# Autodesk Inventor assembly: COMPONENTS
(part 3 of 4)
- C:\Users\rtreacy\Documents\Inventor\SNAP Enclosure 8x10x1.75 Ver1.A\drawings\SNAP Ver2 pack-n-go\Workgroups\NotInProject\INDM9630X305N_L19.ipt
- C:\Users\rtreacy\Documents\Inventor\SNAP Enclosure 8x10x1.75 Ver1.A\drawings\SNAP Ver2 pack-n-go\Workgroups\NotInProject\INDC1608X95L-ALT1_L20.ipt
- C:\Users\rtreacy\Documents\Inventor\SNAP Enclosure 8x10x1.75 Ver1.A\drawings\SNAP Ver2 pack-n-go\Workgroups\NotInProject\INDC1608X95L-ALT1_L21.ipt
- C:\Users\rtreacy\Documents\Inventor\SNAP Enclosure 8x10x1.75 Ver1.A\drawings\SNAP Ver2 pack-n-go\Workgroups\NotInProject\INDC1608X95L-ALT1_L23.ipt
- C:\Users\rtreacy\Documents\Inventor\SNAP Enclosure 8x10x1.75 Ver1.A\drawings\SNAP Ver2 pack-n-go\Workgroups\NotInProject\INDC1608X95L-ALT1_L22.ipt
- C:\Users\rtreacy\Documents\Inventor\SNAP Enclosure 8x10x1.75 Ver1.A\drawings\SNAP Ver2 pack-n-go\Workgroups\NotInProject\INDM5551X200N_L24.ipt
- C:\Users\rtreacy\Documents\Inventor\SNAP Enclosure 8x10x1.75 Ver1.A\drawings\SNAP Ver2 pack-n-go\Workgroups\NotInProject\INDM5551X200N_L25.ipt
- C:\Users\rtreacy\Documents\Inventor\SNAP Enclosure 8x10x1.75 Ver1.A\drawings\SNAP Ver2 pack-n-go\Workgroups\NotInProject\INDM5551X200N_L26.ipt
- C:\Users\rtreacy\Documents\Inventor\SNAP Enclosure 8x10x1.75 Ver1.A\drawings\SNAP Ver2 pack-n-go\Workgroups\NotInProject\INDM5551X200N_L27.ipt
- C:\Users\rtreacy\Documents\Inventor\SNAP Enclosure 8x10x1.75 Ver1.A\drawings\SNAP Ver2 pack-n-go\Workgroups\NotInProject\RESC1005X35N_R443.ipt
- C:\Users\rtreacy\Documents\Inventor\SNAP Enclosure 8x10x1.75 Ver1.A\drawings\SNAP Ver2 pack-n-go\Workgroups\NotInProject\RESC1005X35N_R442.ipt
- C:\Users\rtreacy\Documents\Inventor\SNAP Enclosure 8x10x1.75 Ver1.A\drawings\SNAP Ver2 pack-n-go\Workgroups\NotInProject\RESC1005X35N_R438.ipt
- C:\Users\rtreacy\Documents\Inventor\SNAP Enclosure 8x10x1.75 Ver1.A\drawings\SNAP Ver2 pack-n-go\Workgroups\NotInProject\RESC1005X35N_R437.ipt
- C:\Users\rtreacy\Documents\Inventor\SNAP Enclosure 8x10x1.75 Ver1.A\drawings\SNAP Ver2 pack-n-go\Workgroups\NotInProject\RESC1005X35N_R436.ipt
- C:\Users\rtreacy\Documents\Inventor\SNAP Enclosure 8x10x1.75 Ver1.A\drawings\SNAP Ver2 pack-n-go\Workgroups\NotInProject\RESC1005X35N_R434.ipt
- C:\Users\rtreacy\Documents\Inventor\SNAP Enclosure 8x10x1.75 Ver1.A\drawings\SNAP Ver2 pack-n-go\Workgroups\NotInProject\RESC1005X35N_R114.ipt
- C:\Users\rtreacy\Documents\Inventor\SNAP Enclosure 8x10x1.75 Ver1.A\drawings\SNAP Ver2 pack-n-go\Workgroups\NotInProject\RESC1005X35N_R133.ipt
- C:\Users\rtreacy\Documents\Inventor\SNAP Enclosure 8x10x1.75 Ver1.A\drawings\SNAP Ver2 pack-n-go\Workgroups\NotInProject\RESC1005X35N_R135.ipt
- C:\Users\rtreacy\Documents\Inventor\SNAP Enclosure 8x10x1.75 Ver1.A\drawings\SNAP Ver2 pack-n-go\Workgroups\NotInProject\RESC1005X35N_R139.ipt
- C:\Users\rtreacy\Documents\Inventor\SNAP Enclosure 8x10x1.75 Ver1.A\drawings\SNAP Ver2 pack-n-go\Workgroups\NotInProject\RESC1005X35N_R432.ipt
- C:\Users\rtreacy\Documents\Inventor\SNAP Enclosure 8x10x1.75 Ver1.A\drawings\SNAP Ver2 pack-n-go\Workgroups\NotInProject\RESC1005X35N_R431.ipt
- C:\Users\rtreacy\Documents\Inventor\SNAP Enclosure 8x10x1.75 Ver1.A\drawings\SNAP Ver2 pack-n-go\Workgroups\NotInProject\RESC1005X35N_R427.ipt
- C:\Users\rtreacy\Documents\Inventor\SNAP Enclosure 8x10x1.75 Ver1.A\drawings\SNAP Ver2 pack-n-go\Workgroups\NotInProject\RESC1005X35N_R426.ipt
- C:\Users\rtreacy\Documents\Inventor\SNAP Enclosure 8x10x1.75 Ver1.A\drawings\SNAP Ver2 pack-n-go\Workgroups\NotInProject\RESC1005X35N_R424.ipt
- C:\Users\rtreacy\Documents\Inventor\SNAP Enclosure 8x10x1.75 Ver1.A\drawings\SNAP Ver2 pack-n-go\Workgroups\NotInProject\RESC1005X35N_R423.ipt
- C:\Users\rtreacy\Documents\Inventor\SNAP Enclosure 8x10x1.75 Ver1.A\drawings\SNAP Ver2 pack-n-go\Workgroups\NotInProject\RESC1005X35N_R421.ipt
- C:\Users\rtreacy\Documents\Inventor\SNAP Enclosure 8x10x1.75 Ver1.A\drawings\SNAP Ver2 pack-n-go\Workgroups\NotInProject\RESC1005X35N_R420.ipt
- C:\Users\rtreacy\Documents\Inventor\SNAP Enclosure 8x10x1.75 Ver1.A\drawings\SNAP Ver2 pack-n-go\Workgroups\NotInProject\RESC1005X35N_R433.ipt
- C:\Users\rtreacy\Documents\Inventor\SNAP Enclosure 8x10x1.75 Ver1.A\drawings\SNAP Ver2 pack-n-go\Workgroups\NotInProject\RESC1005X35N_R428.ipt
- C:\Users\rtreacy\Documents\Inventor\SNAP Enclosure 8x10x1.75 Ver1.A\drawings\SNAP Ver2 pack-n-go\Workgroups\NotInProject\RESC1005X35N_R425.ipt
- C:\Users\rtreacy\Documents\Inventor\SNAP Enclosure 8x10x1.75 Ver1.A\drawings\SNAP Ver2 pack-n-go\Workgroups\NotInProject\RESC1005X35N_R422.ipt
- C:\Users\rtreacy\Documents\Inventor\SNAP Enclosure 8x10x1.75 Ver1.A\drawings\SNAP Ver2 pack-n-go\Workgroups\NotInProject\RESC1005X35N_R1.ipt
- C:\Users\rtreacy\Documents\Inventor\SNAP Enclosure 8x10x1.75 Ver1.A\drawings\SNAP Ver2 pack-n-go\Workgroups\NotInProject\RESC1005X35N_R12.ipt
- C:\Users\rtreacy\Documents\Inventor\SNAP Enclosure 8x10x1.75 Ver1.A\drawings\SNAP Ver2 pack-n-go\Workgroups\NotInProject\RESC1005X35N_R13.ipt
- C:\Users\rtreacy\Documents\Inventor\SNAP Enclosure 8x10x1.75 Ver1.A\drawings\SNAP Ver2 pack-n-go\Workgroups\NotInProject\RESC1005X35N_R16.ipt
- C:\Users\rtreacy\Documents\Inventor\SNAP Enclosure 8x10x1.75 Ver1.A\drawings\SNAP Ver2 pack-n-go\Workgroups\NotInProject\RESC1005X35N_R21.ipt
- C:\Users\rtreacy\Documents\Inventor\SNAP Enclosure 8x10x1.75 Ver1.A\drawings\SNAP Ver2 pack-n-go\Workgroups\NotInProject\RESC1005X35N_R25.ipt
- C:\Users\rtreacy\Documents\Inventor\SNAP Enclosure 8x10x1.75 Ver1.A\drawings\SNAP Ver2 pack-n-go\Workgroups\NotInProject\RESC1005X35N_R26.ipt
- C:\Users\rtreacy\Documents\Inventor\SNAP Enclosure 8x10x1.75 Ver1.A\drawings\SNAP Ver2 pack-n-go\Workgroups\NotInProject\RESC1005X35N_R28.ipt
- C:\Users\rtreacy\Documents\Inventor\SNAP Enclosure 8x10x1.75 Ver1.A\drawings\SNAP Ver2 pack-n-go\Workgroups\NotInProject\RESC1005X35N_R29.ipt
- C:\Users\rtreacy\Documents\Inventor\SNAP Enclosure 8x10x1.75 Ver1.A\drawings\SNAP Ver2 pack-n-go\Workgroups\NotInProject\RESC1005X35N_R32.ipt
- C:\Users\rtreacy\Documents\Inventor\SNAP Enclosure 8x10x1.75 Ver1.A\drawings\SNAP Ver2 pack-n-go\Workgroups\NotInProject\RESC1005X35N_R33.ipt
- C:\Users\rtreacy\Documents\Inventor\SNAP Enclosure 8x10x1.75 Ver1.A\drawings\SNAP Ver2 pack-n-go\Workgroups\NotInProject\RESC1005X35N_R36.ipt
- C:\Users\rtreacy\Documents\Inventor\SNAP Enclosure 8x10x1.75 Ver1.A\drawings\SNAP Ver2 pack-n-go\Workgroups\NotInProject\RESC1005X35N_R41.ipt
- C:\Users\rtreacy\Documents\Inventor\SNAP Enclosure 8x10x1.75 Ver1.A\drawings\SNAP Ver2 pack-n-go\Workgroups\NotInProject\RESC1005X35N_R45.ipt
- C:\Users\rtreacy\Documents\Inventor\SNAP Enclosure 8x10x1.75 Ver1.A\drawings\SNAP Ver2 pack-n-go\Workgroups\NotInProject\RESC1005X35N_R46.ipt
- C:\Users\rtreacy\Documents\Inventor\SNAP Enclosure 8x10x1.75 Ver1.A\drawings\SNAP Ver2 pack-n-go\Workgroups\NotInProject\RESC1005X35N_R48.ipt
- C:\Users\rtreacy\Documents\Inventor\SNAP Enclosure 8x10x1.75 Ver1.A\drawings\SNAP Ver2 pack-n-go\Workgroups\NotInProject\RESC1005X35N_R49.ipt
- C:\Users\rtreacy\Documents\Inventor\SNAP Enclosure 8x10x1.75 Ver1.A\drawings\SNAP Ver2 pack-n-go\Workgroups\NotInProject\RESC1005X35N_R5.ipt
- C:\Users\rtreacy\Documents\Inventor\SNAP Enclosure 8x10x1.75 Ver1.A\drawings\SNAP Ver2 pack-n-go\Workgroups\NotInProject\RESC1005X35N_R52.ipt
- C:\Users\rtreacy\Documents\Inventor\SNAP Enclosure 8x10x1.75 Ver1.A\drawings\SNAP Ver2 pack-n-go\Workgroups\NotInProject\RESC1005X35N_R53.ipt
- C:\Users\rtreacy\Documents\Inventor\SNAP Enclosure 8x10x1.75 Ver1.A\drawings\SNAP Ver2 pack-n-go\Workgroups\NotInProject\RESC1005X35N_R56.ipt
- C:\Users\rtreacy\Documents\Inventor\SNAP Enclosure 8x10x1.75 Ver1.A\drawings\SNAP Ver2 pack-n-go\Workgroups\NotInProject\RESC1005X35N_R6.ipt
- C:\Users\rtreacy\Documents\Inventor\SNAP Enclosure 8x10x1.75 Ver1.A\drawings\SNAP Ver2 pack-n-go\Workgroups\NotInProject\RESC1005X35N_R8.ipt
- C:\Users\rtreacy\Documents\Inventor\SNAP Enclosure 8x10x1.75 Ver1.A\drawings\SNAP Ver2 pack-n-go\Workgroups\NotInProject\RESC1005X35N_R9.ipt
- C:\Users\rtreacy\Documents\Inventor\SNAP Enclosure 8x10x1.75 Ver1.A\drawings\SNAP Ver2 pack-n-go\Workgroups\NotInProject\RESC1005X35N_R10.ipt
- C:\Users\rtreacy\Documents\Inventor\SNAP Enclosure 8x10x1.75 Ver1.A\drawings\SNAP Ver2 pack-n-go\Workgroups\NotInProject\RESC1005X35N_R14.ipt
- C:\Users\rtreacy\Documents\Inventor\SNAP Enclosure 8x10x1.75 Ver1.A\drawings\SNAP Ver2 pack-n-go\Workgroups\NotInProject\RESC1005X35N_R2.ipt
- C:\Users\rtreacy\Documents\Inventor\SNAP Enclosure 8x10x1.75 Ver1.A\drawings\SNAP Ver2 pack-n-go\Workgroups\NotInProject\RESC1005X35N_R22.ipt
- C:\Users\rtreacy\Documents\Inventor\SNAP Enclosure 8x10x1.75 Ver1.A\drawings\SNAP Ver2 pack-n-go\Workgroups\NotInProject\RESC1005X35N_R24.ipt
- C:\Users\rtreacy\Documents\Inventor\SNAP Enclosure 8x10x1.75 Ver1.A\drawings\SNAP Ver2 pack-n-go\Workgroups\NotInProject\RESC1005X35N_R30.ipt
- C:\Users\rtreacy\Documents\Inventor\SNAP Enclosure 8x10x1.75 Ver1.A\drawings\SNAP Ver2 pack-n-go\Workgroups\NotInProject\RESC1005X35N_R34.ipt
- C:\Users\rtreacy\Documents\Inventor\SNAP Enclosure 8x10x1.75 Ver1.A\drawings\SNAP Ver2 pack-n-go\Workgroups\NotInProject\RESC1005X35N_R4.ipt
- C:\Users\rtreacy\Documents\Inventor\SNAP Enclosure 8x10x1.75 Ver1.A\drawings\SNAP Ver2 pack-n-go\Workgroups\NotInProject\RESC1005X35N_R42.ipt
- C:\Users\rtreacy\Documents\Inventor\SNAP Enclosure 8x10x1.75 Ver1.A\drawings\SNAP Ver2 pack-n-go\Workgroups\NotInProject\RESC1005X35N_R44.ipt
- C:\Users\rtreacy\Documents\Inventor\SNAP Enclosure 8x10x1.75 Ver1.A\drawings\SNAP Ver2 pack-n-go\Workgroups\NotInProject\RESC1005X35N_R50.ipt
- C:\Users\rtreacy\Documents\Inventor\SNAP Enclosure 8x10x1.75 Ver1.A\drawings\SNAP Ver2 pack-n-go\Workgroups\NotInProject\RESC1005X35N_R54.ipt
- C:\Users\rtreacy\Documents\Inventor\SNAP Enclosure 8x10x1.75 Ver1.A\drawings\SNAP Ver2 pack-n-go\Workgroups\NotInProject\RESC1005X35N_R100.ipt
- C:\Users\rtreacy\Documents\Inventor\SNAP Enclosure 8x10x1.75 Ver1.A\drawings\SNAP Ver2 pack-n-go\Workgroups\NotInProject\RESC1005X35N_R102.ipt
- C:\Users\rtreacy\Documents\Inventor\SNAP Enclosure 8x10x1.75 Ver1.A\drawings\SNAP Ver2 pack-n-go\Workgroups\NotInProject\RESC1005X35N_R103.ipt
- C:\Users\rtreacy\Documents\Inventor\SNAP Enclosure 8x10x1.75 Ver1.A\drawings\SNAP Ver2 pack-n-go\Workgroups\NotInProject\RESC1005X35N_R104.ipt
- C:\Users\rtreacy\Documents\Inventor\SNAP Enclosure 8x10x1.75 Ver1.A\drawings\SNAP Ver2 pack-n-go\Workgroups\NotInProject\RESC1005X35N_R105.ipt
- C:\Users\rtreacy\Documents\Inventor\SNAP Enclosure 8x10x1.75 Ver1.A\drawings\SNAP Ver2 pack-n-go\Workgroups\NotInProject\RESC1005X35N_R106.ipt
- C:\Users\rtreacy\Documents\Inventor\SNAP Enclosure 8x10x1.75 Ver1.A\drawings\SNAP Ver2 pack-n-go\Workgroups\NotInProject\RESC1005X35N_R96.ipt
- C:\Users\rtreacy\Documents\Inventor\SNAP Enclosure 8x10x1.75 Ver1.A\drawings\SNAP Ver2 pack-n-go\Workgroups\NotInProject\RESC1005X35N_R97.ipt
- C:\Users\rtreacy\Documents\Inventor\SNAP Enclosure 8x10x1.75 Ver1.A\drawings\SNAP Ver2 pack-n-go\Workgroups\NotInProject\RESC1005X35N_R109.ipt
- C:\Users\rtreacy\Documents\Inventor\SNAP Enclosure 8x10x1.75 Ver1.A\drawings\SNAP Ver2 pack-n-go\Workgroups\NotInProject\RESC1005X35N_R140.ipt
- C:\Users\rtreacy\Documents\Inventor\SNAP Enclosure 8x10x1.75 Ver1.A\drawings\SNAP Ver2 pack-n-go\Workgroups\NotInProject\RESC1005X35N_R145.ipt
- C:\Users\rtreacy\Documents\Inventor\SNAP Enclosure 8x10x1.75 Ver1.A\drawings\SNAP Ver2 pack-n-go\Workgroups\NotInProject\RESC1005X35N_R146.ipt
- C:\Users\rtreacy\Documents\Inventor\SNAP Enclosure 8x10x1.75 Ver1.A\drawings\SNAP Ver2 pack-n-go\Workgroups\NotInProject\RESC1005X35N_R147.ipt
- C:\Users\rtreacy\Documents\Inventor\SNAP Enclosure 8x10x1.75 Ver1.A\drawings\SNAP Ver2 pack-n-go\Workgroups\NotInProject\RESC1005X35N_R148.ipt
- C:\Users\rtreacy\Documents\Inventor\SNAP Enclosure 8x10x1.75 Ver1.A\drawings\SNAP Ver2 pack-n-go\Workgroups\NotInProject\RESC1005X35N_R154.ipt
- C:\Users\rtreacy\Documents\Inventor\SNAP Enclosure 8x10x1.75 Ver1.A\drawings\SNAP Ver2 pack-n-go\Workgroups\NotInProject\RESC1005X35N_R157.ipt
- C:\Users\rtreacy\Documents\Inventor\SNAP Enclosure 8x10x1.75 Ver1.A\drawings\SNAP Ver2 pack-n-go\Workgroups\NotInProject\RESC1005X35N_R158.ipt
- C:\Users\rtreacy\Documents\Inventor\SNAP Enclosure 8x10x1.75 Ver1.A\drawings\SNAP Ver2 pack-n-go\Workgroups\NotInProject\RESC1005X35N_R159.ipt
- C:\Users\rtreacy\Documents\Inventor\SNAP Enclosure 8x10x1.75 Ver1.A\drawings\SNAP Ver2 pack-n-go\Workgroups\NotInProject\RESC1005X35N_R160.ipt
- C:\Users\rtreacy\Documents\Inventor\SNAP Enclosure 8x10x1.75 Ver1.A\drawings\SNAP Ver2 pack-n-go\Workgroups\NotInProject\RESC1005X35N_R161.ipt
- C:\Users\rtreacy\Documents\Inventor\SNAP Enclosure 8x10x1.75 Ver1.A\drawings\SNAP Ver2 pack-n-go\Workgroups\NotInProject\RESC1005X35N_R162.ipt
- C:\Users\rtreacy\Documents\Inventor\SNAP Enclosure 8x10x1.75 Ver1.A\drawings\SNAP Ver2 pack-n-go\Workgroups\NotInProject\RESC1005X35N_R163.ipt
- C:\Users\rtreacy\Documents\Inventor\SNAP Enclosure 8x10x1.75 Ver1.A\drawings\SNAP Ver2 pack-n-go\Workgroups\NotInProject\RESC1005X35N_R164.ipt
- C:\Users\rtreacy\Documents\Inventor\SNAP Enclosure 8x10x1.75 Ver1.A\drawings\SNAP Ver2 pack-n-go\Workgroups\NotInProject\RESC1005X35N_R194.ipt
- C:\Users\rtreacy\Documents\Inventor\SNAP Enclosure 8x10x1.75 Ver1.A\drawings\SNAP Ver2 pack-n-go\Workgroups\NotInProject\RESC1005X35N_R195.ipt
- C:\Users\rtreacy\Documents\Inventor\SNAP Enclosure 8x10x1.75 Ver1.A\drawings\SNAP Ver2 pack-n-go\Workgroups\NotInProject\RESC1005X35N_R196.ipt
- C:\Users\rtreacy\Documents\Inventor\SNAP Enclosure 8x10x1.75 Ver1.A\drawings\SNAP Ver2 pack-n-go\Workgroups\NotInProject\RESC1005X35N_R201.ipt
- C:\Users\rtreacy\Documents\Inventor\SNAP Enclosure 8x10x1.75 Ver1.A\drawings\SNAP Ver2 pack-n-go\Workgroups\NotInProject\RESC1005X35N_R202.ipt
- C:\Users\rtreacy\Documents\Inventor\SNAP Enclosure 8x10x1.75 Ver1.A\drawings\SNAP Ver2 pack-n-go\Workgroups\NotInProject\RESC1005X35N_R203.ipt
- C:\Users\rtreacy\Documents\Inventor\SNAP Enclosure 8x10x1.75 Ver1.A\drawings\SNAP Ver2 pack-n-go\Workgroups\NotInProject\RESC1005X35N_R204.ipt
- C:\Users\rtreacy\Documents\Inventor\SNAP Enclosure 8x10x1.75 Ver1.A\drawings\SNAP Ver2 pack-n-go\Workgroups\NotInProject\RESC1005X35N_R205.ipt
- C:\Users\rtreacy\Documents\Inventor\SNAP Enclosure 8x10x1.75 Ver1.A\drawings\SNAP Ver2 pack-n-go\Workgroups\NotInProject\RESC1005X35N_R206.ipt
- C:\Users\rtreacy\Documents\Inventor\SNAP Enclosure 8x10x1.75 Ver1.A\drawings\SNAP Ver2 pack-n-go\Workgroups\NotInProject\RESC1005X35N_R207.ipt
- C:\Users\rtreacy\Documents\Inventor\SNAP Enclosure 8x10x1.75 Ver1.A\drawings\SNAP Ver2 pack-n-go\Workgroups\NotInProject\RESC1005X35N_R208.ipt
- C:\Users\rtreacy\Documents\Inventor\SNAP Enclosure 8x10x1.75 Ver1.A\drawings\SNAP Ver2 pack-n-go\Workgroups\NotInProject\RESC1005X35N_R210.ipt
- C:\Users\rtreacy\Documents\Inventor\SNAP Enclosure 8x10x1.75 Ver1.A\drawings\SNAP Ver2 pack-n-go\Workgroups\NotInProject\RESC1005X35N_R211.ipt
- C:\Users\rtreacy\Documents\Inventor\SNAP Enclosure 8x10x1.75 Ver1.A\drawings\SNAP Ver2 pack-n-go\Workgroups\NotInProject\RESC1005X35N_R212.ipt
- C:\Users\rtreacy\Documents\Inventor\SNAP Enclosure 8x10x1.75 Ver1.A\drawings\SNAP Ver2 pack-n-go\Workgroups\NotInProject\RESC1005X35N_R213.ipt
- C:\Users\rtreacy\Documents\Inventor\SNAP Enclosure 8x10x1.75 Ver1.A\drawings\SNAP Ver2 pack-n-go\Workgroups\NotInProject\RESC1005X35N_R214.ipt
- C:\Users\rtreacy\Documents\Inventor\SNAP Enclosure 8x10x1.75 Ver1.A\drawings\SNAP Ver2 pack-n-go\Workgroups\NotInProject\RESC1005X35N_R215.ipt
- C:\Users\rtreacy\Documents\Inventor\SNAP Enclosure 8x10x1.75 Ver1.A\drawings\SNAP Ver2 pack-n-go\Workgroups\NotInProject\RESC1005X35N_R216.ipt
- C:\Users\rtreacy\Documents\Inventor\SNAP Enclosure 8x10x1.75 Ver1.A\drawings\SNAP Ver2 pack-n-go\Workgroups\NotInProject\RESC1005X35N_R217.ipt
- C:\Users\rtreacy\Documents\Inventor\SNAP Enclosure 8x10x1.75 Ver1.A\drawings\SNAP Ver2 pack-n-go\Workgroups\NotInProject\RESC1005X35N_R218.ipt
- C:\Users\rtreacy\Documents\Inventor\SNAP Enclosure 8x10x1.75 Ver1.A\drawings\SNAP Ver2 pack-n-go\Workgroups\NotInProject\RESC1005X35N_R219.ipt
- C:\Users\rtreacy\Documents\Inventor\SNAP Enclosure 8x10x1.75 Ver1.A\drawings\SNAP Ver2 pack-n-go\Workgroups\NotInProject\RESC1005X35N_R221.ipt
- C:\Users\rtreacy\Documents\Inventor\SNAP Enclosure 8x10x1.75 Ver1.A\drawings\SNAP Ver2 pack-n-go\Workgroups\NotInProject\RESC1005X35N_R222.ipt
- C:\Users\rtreacy\Documents\Inventor\SNAP Enclosure 8x10x1.75 Ver1.A\drawings\SNAP Ver2 pack-n-go\Workgroups\NotInProject\RESC1005X35N_R223.ipt
- C:\Users\rtreacy\Documents\Inventor\SNAP Enclosure 8x10x1.75 Ver1.A\drawings\SNAP Ver2 pack-n-go\Workgroups\NotInProject\RESC1005X35N_R224.ipt
- C:\Users\rtreacy\Documents\Inventor\SNAP Enclosure 8x10x1.75 Ver1.A\drawings\SNAP Ver2 pack-n-go\Workgroups\NotInProject\RESC1005X35N_R226.ipt
- C:\Users\rtreacy\Documents\Inventor\SNAP Enclosure 8x10x1.75 Ver1.A\drawings\SNAP Ver2 pack-n-go\Workgroups\NotInProject\RESC1005X35N_R227.ipt
- C:\Users\rtreacy\Documents\Inventor\SNAP Enclosure 8x10x1.75 Ver1.A\drawings\SNAP Ver2 pack-n-go\Workgroups\NotInProject\RESC1005X35N_R11.ipt
- C:\Users\rtreacy\Documents\Inventor\SNAP Enclosure 8x10x1.75 Ver1.A\drawings\SNAP Ver2 pack-n-go\Workgroups\NotInProject\RESC1005X35N_R15.ipt
- C:\Users\rtreacy\Documents\Inventor\SNAP Enclosure 8x10x1.75 Ver1.A\drawings\SNAP Ver2 pack-n-go\Workgroups\NotInProject\RESC1005X35N_R23.ipt
- C:\Users\rtreacy\Documents\Inventor\SNAP Enclosure 8x10x1.75 Ver1.A\drawings\SNAP Ver2 pack-n-go\Workgroups\NotInProject\RESC1005X35N_R27.ipt
- C:\Users\rtreacy\Documents\Inventor\SNAP Enclosure 8x10x1.75 Ver1.A\drawings\SNAP Ver2 pack-n-go\Workgroups\NotInProject\RESC1005X35N_R3.ipt
- C:\Users\rtreacy\Documents\Inventor\SNAP Enclosure 8x10x1.75 Ver1.A\drawings\SNAP Ver2 pack-n-go\Workgroups\NotInProject\RESC1005X35N_R31.ipt
- C:\Users\rtreacy\Documents\Inventor\SNAP Enclosure 8x10x1.75 Ver1.A\drawings\SNAP Ver2 pack-n-go\Workgroups\NotInProject\RESC1005X35N_R35.ipt
- C:\Users\rtreacy\Documents\Inventor\SNAP Enclosure 8x10x1.75 Ver1.A\drawings\SNAP Ver2 pack-n-go\Workgroups\NotInProject\RESC1005X35N_R43.ipt
- C:\Users\rtreacy\Documents\Inventor\SNAP Enclosure 8x10x1.75 Ver1.A\drawings\SNAP Ver2 pack-n-go\Workgroups\NotInProject\RESC1005X35N_R47.ipt
- C:\Users\rtreacy\Documents\Inventor\SNAP Enclosure 8x10x1.75 Ver1.A\drawings\SNAP Ver2 pack-n-go\Workgroups\NotInProject\RESC1005X35N_R51.ipt
- C:\Users\rtreacy\Documents\Inventor\SNAP Enclosure 8x10x1.75 Ver1.A\drawings\SNAP Ver2 pack-n-go\Workgroups\NotInProject\RESC1005X35N_R55.ipt
- C:\Users\rtreacy\Documents\Inventor\SNAP Enclosure 8x10x1.75 Ver1.A\drawings\SNAP Ver2 pack-n-go\Workgroups\NotInProject\RESC1005X35N_R7.ipt
- C:\Users\rtreacy\Documents\Inventor\SNAP Enclosure 8x10x1.75 Ver1.A\drawings\SNAP Ver2 pack-n-go\Workgroups\NotInProject\RESC1005X35N_R110.ipt
- C:\Users\rtreacy\Documents\Inventor\SNAP Enclosure 8x10x1.75 Ver1.A\drawings\SNAP Ver2 pack-n-go\Workgroups\NotInProject\RESC1005X35N_R112.ipt
- C:\Users\rtreacy\Documents\Inventor\SNAP Enclosure 8x10x1.75 Ver1.A\drawings\SNAP Ver2 pack-n-go\Workgroups\NotInProject\RESC1005X35N_R113.ipt
- C:\Users\rtreacy\Documents\Inventor\SNAP Enclosure 8x10x1.75 Ver1.A\drawings\SNAP Ver2 pack-n-go\Workgroups\NotInProject\RESC1005X35N_R115.ipt
- C:\Users\rtreacy\Documents\Inventor\SNAP Enclosure 8x10x1.75 Ver1.A\drawings\SNAP Ver2 pack-n-go\Workgroups\NotInProject\RESC1005X35N_R116.ipt
- C:\Users\rtreacy\Documents\Inventor\SNAP Enclosure 8x10x1.75 Ver1.A\drawings\SNAP Ver2 pack-n-go\Workgroups\NotInProject\RESC1005X35N_R120.ipt
- C:\Users\rtreacy\Documents\Inventor\SNAP Enclosure 8x10x1.75 Ver1.A\drawings\SNAP Ver2 pack-n-go\Workgroups\NotInProject\RESC1005X35N_R124.ipt
- C:\Users\rtreacy\Documents\Inventor\SNAP Enclosure 8x10x1.75 Ver1.A\drawings\SNAP Ver2 pack-n-go\Workgroups\NotInProject\RESC1005X35N_R111.ipt
- C:\Users\rtreacy\Documents\Inventor\SNAP Enclosure 8x10x1.75 Ver1.A\drawings\SNAP Ver2 pack-n-go\Workgroups\NotInProject\RESC1005X35N_R117.ipt
- C:\Users\rtreacy\Documents\Inventor\SNAP Enclosure 8x10x1.75 Ver1.A\drawings\SNAP Ver2 pack-n-go\Workgroups\NotInProject\RESC1005X35N_R119.ipt
- C:\Users\rtreacy\Documents\Inventor\SNAP Enclosure 8x10x1.75 Ver1.A\drawings\SNAP Ver2 pack-n-go\Workgroups\NotInProject\RESC1005X35N_R123.ipt
- C:\Users\rtreacy\Documents\Inventor\SNAP Enclosure 8x10x1.75 Ver1.A\drawings\SNAP Ver2 pack-n-go\Workgroups\NotInProject\RESC1005X35N_R130.ipt
- C:\Users\rtreacy\Documents\Inventor\SNAP Enclosure 8x10x1.75 Ver1.A\drawings\SNAP Ver2 pack-n-go\Workgroups\NotInProject\RESC1005X35N_R132.ipt
- C:\Users\rtreacy\Documents\Inventor\SNAP Enclosure 8x10x1.75 Ver1.A\drawings\SNAP Ver2 pack-n-go\Workgroups\NotInProject\RESC1005X35N_R134.ipt
- C:\Users\rtreacy\Documents\Inventor\SNAP Enclosure 8x10x1.75 Ver1.A\drawings\SNAP Ver2 pack-n-go\Workgroups\NotInProject\RESC1005X35N_R137.ipt
- C:\Users\rtreacy\Documents\Inventor\SNAP Enclosure 8x10x1.75 Ver1.A\drawings\SNAP Ver2 pack-n-go\Workgroups\NotInProject\RESC1005X35N_R170.ipt
- C:\Users\rtreacy\Documents\Inventor\SNAP Enclosure 8x10x1.75 Ver1.A\drawings\SNAP Ver2 pack-n-go\Workgroups\NotInProject\RESC1005X35N_R171.ipt
- C:\Users\rtreacy\Documents\Inventor\SNAP Enclosure 8x10x1.75 Ver1.A\drawings\SNAP Ver2 pack-n-go\Workgroups\NotInProject\RESC1005X35N_R175.ipt
- C:\Users\rtreacy\Documents\Inventor\SNAP Enclosure 8x10x1.75 Ver1.A\drawings\SNAP Ver2 pack-n-go\Workgroups\NotInProject\RESC1005X35N_R178.ipt
- C:\Users\rtreacy\Documents\Inventor\SNAP Enclosure 8x10x1.75 Ver1.A\drawings\SNAP Ver2 pack-n-go\Workgroups\NotInProject\RESC1005X35N_R183.ipt
- C:\Users\rtreacy\Documents\Inventor\SNAP Enclosure 8x10x1.75 Ver1.A\drawings\SNAP Ver2 pack-n-go\Workgroups\NotInProject\RESC1005X35N_R184.ipt
- C:\Users\rtreacy\Documents\Inventor\SNAP Enclosure 8x10x1.75 Ver1.A\drawings\SNAP Ver2 pack-n-go\Workgroups\NotInProject\RESC1005X35N_R188.ipt
- C:\Users\rtreacy\Documents\Inventor\SNAP Enclosure 8x10x1.75 Ver1.A\drawings\SNAP Ver2 pack-n-go\Workgroups\NotInProject\RESC1005X35N_R191.ipt
- C:\Users\rtreacy\Documents\Inventor\SNAP Enclosure 8x10x1.75 Ver1.A\drawings\SNAP Ver2 pack-n-go\Workgroups\NotInProject\RESC1005X35N_R118.ipt
- C:\Users\rtreacy\Documents\Inventor\SNAP Enclosure 8x10x1.75 Ver1.A\drawings\SNAP Ver2 pack-n-go\Workgroups\NotInProject\RESC1005X35N_R121.ipt
- C:\Users\rtreacy\Documents\Inventor\SNAP Enclosure 8x10x1.75 Ver1.A\drawings\SNAP Ver2 pack-n-go\Workgroups\NotInProject\RESC1005X35N_R126.ipt
- C:\Users\rtreacy\Documents\Inventor\SNAP Enclosure 8x10x1.75 Ver1.A\drawings\SNAP Ver2 pack-n-go\Workgroups\NotInProject\RESC1005X35N_R131.ipt
- C:\Users\rtreacy\Documents\Inventor\SNAP Enclosure 8x10x1.75 Ver1.A\drawings\SNAP Ver2 pack-n-go\Workgroups\NotInProject\RESC1005X35N_R122.ipt
- C:\Users\rtreacy\Documents\Inventor\SNAP Enclosure 8x10x1.75 Ver1.A\drawings\SNAP Ver2 pack-n-go\Workgroups\NotInProject\RESC1005X35N_R125.ipt
- C:\Users\rtreacy\Documents\Inventor\SNAP Enclosure 8x10x1.75 Ver1.A\drawings\SNAP Ver2 pack-n-go\Workgroups\NotInProject\RESC1005X35N_R138.ipt
- C:\Users\rtreacy\Documents\Inventor\SNAP Enclosure 8x10x1.75 Ver1.A\drawings\SNAP Ver2 pack-n-go\Workgroups\NotInProject\RESC1005X35N_R127.ipt
- C:\Users\rtreacy\Documents\Inventor\SNAP Enclosure 8x10x1.75 Ver1.A\drawings\SNAP Ver2 pack-n-go\Workgroups\NotInProject\RESC1005X35N_R128.ipt
- C:\Users\rtreacy\Documents\Inventor\SNAP Enclosure 8x10x1.75 Ver1.A\drawings\SNAP Ver2 pack-n-go\Workgroups\NotInProject\RESC1005X35N_R166.ipt
- C:\Users\rtreacy\Documents\Inventor\SNAP Enclosure 8x10x1.75 Ver1.A\drawings\SNAP Ver2 pack-n-go\Workgroups\NotInProject\RESC1005X35N_R167.ipt
- C:\Users\rtreacy\Documents\Inventor\SNAP Enclosure 8x10x1.75 Ver1.A\drawings\SNAP Ver2 pack-n-go\Workgroups\NotInProject\RESC1005X35N_R169.ipt
- C:\Users\rtreacy\Documents\Inventor\SNAP Enclosure 8x10x1.75 Ver1.A\drawings\SNAP Ver2 pack-n-go\Workgroups\NotInProject\RESC1005X35N_R172.ipt
- C:\Users\rtreacy\Documents\Inventor\SNAP Enclosure 8x10x1.75 Ver1.A\drawings\SNAP Ver2 pack-n-go\Workgroups\NotInProject\RESC1005X35N_R173.ipt
- C:\Users\rtreacy\Documents\Inventor\SNAP Enclosure 8x10x1.75 Ver1.A\drawings\SNAP Ver2 pack-n-go\Workgroups\NotInProject\RESC1005X35N_R174.ipt
- C:\Users\rtreacy\Documents\Inventor\SNAP Enclosure 8x10x1.75 Ver1.A\drawings\SNAP Ver2 pack-n-go\Workgroups\NotInProject\RESC1005X35N_R176.ipt
- C:\Users\rtreacy\Documents\Inventor\SNAP Enclosure 8x10x1.75 Ver1.A\drawings\SNAP Ver2 pack-n-go\Workgroups\NotInProject\RESC1005X35N_R177.ipt
- C:\Users\rtreacy\Documents\Inventor\SNAP Enclosure 8x10x1.75 Ver1.A\drawings\SNAP Ver2 pack-n-go\Workgroups\NotInProject\RESC1005X35N_R179.ipt
- C:\Users\rtreacy\Documents\Inventor\SNAP Enclosure 8x10x1.75 Ver1.A\drawings\SNAP Ver2 pack-n-go\Workgroups\NotInProject\RESC1005X35N_R180.ipt
- C:\Users\rtreacy\Documents\Inventor\SNAP Enclosure 8x10x1.75 Ver1.A\drawings\SNAP Ver2 pack-n-go\Workgroups\NotInProject\RESC1005X35N_R182.ipt
- C:\Users\rtreacy\Documents\Inventor\SNAP Enclosure 8x10x1.75 Ver1.A\drawings\SNAP Ver2 pack-n-go\Workgroups\NotInProject\RESC1005X35N_R185.ipt
- C:\Users\rtreacy\Documents\Inventor\SNAP Enclosure 8x10x1.75 Ver1.A\drawings\SNAP Ver2 pack-n-go\Workgroups\NotInProject\RESC1005X35N_R186.ipt
- C:\Users\rtreacy\Documents\Inventor\SNAP Enclosure 8x10x1.75 Ver1.A\drawings\SNAP Ver2 pack-n-go\Workgroups\NotInProject\RESC1005X35N_R187.ipt
- C:\Users\rtreacy\Documents\Inventor\SNAP Enclosure 8x10x1.75 Ver1.A\drawings\SNAP Ver2 pack-n-go\Workgroups\NotInProject\RESC1005X35N_R189.ipt
- C:\Users\rtreacy\Documents\Inventor\SNAP Enclosure 8x10x1.75 Ver1.A\drawings\SNAP Ver2 pack-n-go\Workgroups\NotInProject\RESC1005X35N_R190.ipt
- C:\Users\rtreacy\Documents\Inventor\SNAP Enclosure 8x10x1.75 Ver1.A\drawings\SNAP Ver2 pack-n-go\Workgroups\NotInProject\RESC1005X35N_R136.ipt
- C:\Users\rtreacy\Documents\Inventor\SNAP Enclosure 8x10x1.75 Ver1.A\drawings\SNAP Ver2 pack-n-go\Workgroups\NotInProject\RESC1005X35N_R141.ipt
- C:\Users\rtreacy\Documents\Inventor\SNAP Enclosure 8x10x1.75 Ver1.A\drawings\SNAP Ver2 pack-n-go\Workgroups\NotInProject\RESC1005X35N_R142.ipt
- C:\Users\rtreacy\Documents\Inventor\SNAP Enclosure 8x10x1.75 Ver1.A\drawings\SNAP Ver2 pack-n-go\Workgroups\NotInProject\RESC1005X35N_R143.ipt
- C:\Users\rtreacy\Documents\Inventor\SNAP Enclosure 8x10x1.75 Ver1.A\drawings\SNAP Ver2 pack-n-go\Workgroups\NotInProject\RESC1005X35N_R144.ipt
- C:\Users\rtreacy\Documents\Inventor\SNAP Enclosure 8x10x1.75 Ver1.A\drawings\SNAP Ver2 pack-n-go\Workgroups\NotInProject\RESC1005X35N_R197.ipt
- C:\Users\rtreacy\Documents\Inventor\SNAP Enclosure 8x10x1.75 Ver1.A\drawings\SNAP Ver2 pack-n-go\Workgroups\NotInProject\RESC1005X35N_R198.ipt
- C:\Users\rtreacy\Documents\Inventor\SNAP Enclosure 8x10x1.75 Ver1.A\drawings\SNAP Ver2 pack-n-go\Workgroups\NotInProject\RESC1005X35N_R199.ipt
- C:\Users\rtreacy\Documents\Inventor\SNAP Enclosure 8x10x1.75 Ver1.A\drawings\SNAP Ver2 pack-n-go\Workgroups\NotInProject\RESC1005X35N_R200.ipt
- C:\Users\rtreacy\Documents\Inventor\SNAP Enclosure 8x10x1.75 Ver1.A\drawings\SNAP Ver2 pack-n-go\Workgroups\NotInProject\RESC1005X35N_R155.ipt
- C:\Users\rtreacy\Documents\Inventor\SNAP Enclosure 8x10x1.75 Ver1.A\drawings\SNAP Ver2 pack-n-go\Workgroups\NotInProject\RESC1005X35N_R156.ipt
- C:\Users\rtreacy\Documents\Inventor\SNAP Enclosure 8x10x1.75 Ver1.A\drawings\SNAP Ver2 pack-n-go\Workgroups\NotInProject\RESC1005X35N_R225.ipt
- C:\Users\rtreacy\Documents\Inventor\SNAP Enclosure 8x10x1.75 Ver1.A\drawings\SNAP Ver2 pack-n-go\Workgroups\NotInProject\RESC1005X35N_R228.ipt
- C:\Users\rtreacy\Documents\Inventor\SNAP Enclosure 8x10x1.75 Ver1.A\drawings\SNAP Ver2 pack-n-go\Workgroups\NotInProject\RESC1005X35N_R229.ipt
- C:\Users\rtreacy\Documents\Inventor\SNAP Enclosure 8x10x1.75 Ver1.A\drawings\SNAP Ver2 pack-n-go\Workgroups\NotInProject\RESC1005X35N_R230.ipt
- C:\Users\rtreacy\Documents\Inventor\SNAP Enclosure 8x10x1.75 Ver1.A\drawings\SNAP Ver2 pack-n-go\Workgroups\NotInProject\RESC1005X35N_R231.ipt
- C:\Users\rtreacy\Documents\Inventor\SNAP Enclosure 8x10x1.75 Ver1.A\drawings\SNAP Ver2 pack-n-go\Workgroups\NotInProject\RESC1005X35N_R232.ipt
- C:\Users\rtreacy\Documents\Inventor\SNAP Enclosure 8x10x1.75 Ver1.A\drawings\SNAP Ver2 pack-n-go\Workgroups\NotInProject\RESC1005X35N_R233.ipt
- C:\Users\rtreacy\Documents\Inventor\SNAP Enclosure 8x10x1.75 Ver1.A\drawings\SNAP Ver2 pack-n-go\Workgroups\NotInProject\RESC1005X35N_R234.ipt
- C:\Users\rtreacy\Documents\Inventor\SNAP Enclosure 8x10x1.75 Ver1.A\drawings\SNAP Ver2 pack-n-go\Workgroups\NotInProject\RESC1005X35N_R168.ipt
- C:\Users\rtreacy\Documents\Inventor\SNAP Enclosure 8x10x1.75 Ver1.A\drawings\SNAP Ver2 pack-n-go\Workgroups\NotInProject\RESC1005X35N_R181.ipt
- C:\Users\rtreacy\Documents\Inventor\SNAP Enclosure 8x10x1.75 Ver1.A\drawings\SNAP Ver2 pack-n-go\Workgroups\NotInProject\RESC1005X35N_R17.ipt
- C:\Users\rtreacy\Documents\Inventor\SNAP Enclosure 8x10x1.75 Ver1.A\drawings\SNAP Ver2 pack-n-go\Workgroups\NotInProject\RESC1005X35N_R18.ipt
- C:\Users\rtreacy\Documents\Inventor\SNAP Enclosure 8x10x1.75 Ver1.A\drawings\SNAP Ver2 pack-n-go\Workgroups\NotInProject\RESC1005X35N_R37.ipt
- C:\Users\rtreacy\Documents\Inventor\SNAP Enclosure 8x10x1.75 Ver1.A\drawings\SNAP Ver2 pack-n-go\Workgroups\NotInProject\RESC1005X35N_R38.ipt
- C:\Users\rtreacy\Documents\Inventor\SNAP Enclosure 8x10x1.75 Ver1.A\drawings\SNAP Ver2 pack-n-go\Workgroups\NotInProject\RESC1005X35N_R57.ipt
- C:\Users\rtreacy\Documents\Inventor\SNAP Enclosure 8x10x1.75 Ver1.A\drawings\SNAP Ver2 pack-n-go\Workgroups\NotInProject\RESC1005X35N_R58.ipt
- C:\Users\rtreacy\Documents\Inventor\SNAP Enclosure 8x10x1.75 Ver1.A\drawings\SNAP Ver2 pack-n-go\Workgroups\NotInProject\RESC1005X35N_R19.ipt
- C:\Users\rtreacy\Documents\Inventor\SNAP Enclosure 8x10x1.75 Ver1.A\drawings\SNAP Ver2 pack-n-go\Workgroups\NotInProject\RESC1005X35N_R39.ipt
- C:\Users\rtreacy\Documents\Inventor\SNAP Enclosure 8x10x1.75 Ver1.A\drawings\SNAP Ver2 pack-n-go\Workgroups\NotInProject\RESC1005X35N_R59.ipt
- C:\Users\rtreacy\Documents\Inventor\SNAP Enclosure 8x10x1.75 Ver1.A\drawings\SNAP Ver2 pack-n-go\Workgroups\NotInProject\RESC1005X35N_R20.ipt
- C:\Users\rtreacy\Documents\Inventor\SNAP Enclosure 8x10x1.75 Ver1.A\drawings\SNAP Ver2 pack-n-go\Workgroups\NotInProject\RESC1005X35N_R40.ipt
- C:\Users\rtreacy\Documents\Inventor\SNAP Enclosure 8x10x1.75 Ver1.A\drawings\SNAP Ver2 pack-n-go\Workgroups\NotInProject\RESC1005X35N_R60.ipt
- C:\Users\rtreacy\Documents\Inventor\SNAP Enclosure 8x10x1.75 Ver1.A\drawings\SNAP Ver2 pack-n-go\Workgroups\NotInProject\RESC1005X35N_R209.ipt
- C:\Users\rtreacy\Documents\Inventor\SNAP Enclosure 8x10x1.75 Ver1.A\drawings\SNAP Ver2 pack-n-go\Workgroups\NotInProject\RESC1005X35N_R220.ipt
- C:\Users\rtreacy\Documents\Inventor\SNAP Enclosure 8x10x1.75 Ver1.A\drawings\SNAP Ver2 pack-n-go\Workgroups\NotInProject\RESC1005X35N_R61.ipt
- C:\Users\rtreacy\Documents\Inventor\SNAP Enclosure 8x10x1.75 Ver1.A\drawings\SNAP Ver2 pack-n-go\Workgroups\NotInProject\RESC1005X35N_R65.ipt
- C:\Users\rtreacy\Documents\Inventor\SNAP Enclosure 8x10x1.75 Ver1.A\drawings\SNAP Ver2 pack-n-go\Workgroups\NotInProject\RESC1005X35N_R67.ipt
- C:\Users\rtreacy\Documents\Inventor\SNAP Enclosure 8x10x1.75 Ver1.A\drawings\SNAP Ver2 pack-n-go\Workgroups\NotInProject\RESC1005X35N_R62.ipt
- C:\Users\rtreacy\Documents\Inventor\SNAP Enclosure 8x10x1.75 Ver1.A\drawings\SNAP Ver2 pack-n-go\Workgroups\NotInProject\RESC1005X35N_R64.ipt
- C:\Users\rtreacy\Documents\Inventor\SNAP Enclosure 8x10x1.75 Ver1.A\drawings\SNAP Ver2 pack-n-go\Workgroups\NotInProject\RESC1005X35N_R63.ipt
- C:\Users\rtreacy\Documents\Inventor\SNAP Enclosure 8x10x1.75 Ver1.A\drawings\SNAP Ver2 pack-n-go\Workgroups\NotInProject\RESC1005X35N_R66.ipt
- C:\Users\rtreacy\Documents\Inventor\SNAP Enclosure 8x10x1.75 Ver1.A\drawings\SNAP Ver2 pack-n-go\Workgroups\NotInProject\RESC1005X35N_R70.ipt
- C:\Users\rtreacy\Documents\Inventor\SNAP Enclosure 8x10x1.75 Ver1.A\drawings\SNAP Ver2 pack-n-go\Workgroups\NotInProject\RESC1005X35N_R71.ipt
- C:\Users\rtreacy\Documents\Inventor\SNAP Enclosure 8x10x1.75 Ver1.A\drawings\SNAP Ver2 pack-n-go\Workgroups\NotInProject\RESC1005X35N_R72.ipt
- C:\Users\rtreacy\Documents\Inventor\SNAP Enclosure 8x10x1.75 Ver1.A\drawings\SNAP Ver2 pack-n-go\Workgroups\NotInProject\RESC1005X35N_R73.ipt
- C:\Users\rtreacy\Documents\Inventor\SNAP Enclosure 8x10x1.75 Ver1.A\drawings\SNAP Ver2 pack-n-go\Workgroups\NotInProject\RESC1005X35N_R75.ipt
- C:\Users\rtreacy\Documents\Inventor\SNAP Enclosure 8x10x1.75 Ver1.A\drawings\SNAP Ver2 pack-n-go\Workgroups\NotInProject\RESC1005X35N_R76.ipt
- C:\Users\rtreacy\Documents\Inventor\SNAP Enclosure 8x10x1.75 Ver1.A\drawings\SNAP Ver2 pack-n-go\Workgroups\NotInProject\RESC1005X35N_R77.ipt
- C:\Users\rtreacy\Documents\Inventor\SNAP Enclosure 8x10x1.75 Ver1.A\drawings\SNAP Ver2 pack-n-go\Workgroups\NotInProject\RESC1005X35N_R91.ipt
- C:\Users\rtreacy\Documents\Inventor\SNAP Enclosure 8x10x1.75 Ver1.A\drawings\SNAP Ver2 pack-n-go\Workgroups\NotInProject\RESC1005X35N_R92.ipt
- C:\Users\rtreacy\Documents\Inventor\SNAP Enclosure 8x10x1.75 Ver1.A\drawings\SNAP Ver2 pack-n-go\Workgroups\NotInProject\RESC1005X35N_R94.ipt
- C:\Users\rtreacy\Documents\Inventor\SNAP Enclosure 8x10x1.75 Ver1.A\drawings\SNAP Ver2 pack-n-go\Workgroups\NotInProject\RESC1005X35N_R95.ipt
- C:\Users\rtreacy\Documents\Inventor\SNAP Enclosure 8x10x1.75 Ver1.A\drawings\SNAP Ver2 pack-n-go\Workgroups\NotInProject\RESC1005X35N_R80.ipt
- C:\Users\rtreacy\Documents\Inventor\SNAP Enclosure 8x10x1.75 Ver1.A\drawings\SNAP Ver2 pack-n-go\Workgroups\NotInProject\RESC1005X35N_R81.ipt
- C:\Users\rtreacy\Documents\Inventor\SNAP Enclosure 8x10x1.75 Ver1.A\drawings\SNAP Ver2 pack-n-go\Workgroups\NotInProject\RESC1005X35N_R82.ipt
- C:\Users\rtreacy\Documents\Inventor\SNAP Enclosure 8x10x1.75 Ver1.A\drawings\SNAP Ver2 pack-n-go\Workgroups\NotInProject\RESC1005X35N_R83.ipt
- C:\Users\rtreacy\Documents\Inventor\SNAP Enclosure 8x10x1.75 Ver1.A\drawings\SNAP Ver2 pack-n-go\Workgroups\NotInProject\RESC1005X35N_R84.ipt
- C:\Users\rtreacy\Documents\Inventor\SNAP Enclosure 8x10x1.75 Ver1.A\drawings\SNAP Ver2 pack-n-go\Workgroups\NotInProject\RESC1005X35N_R86.ipt
- C:\Users\rtreacy\Documents\Inventor\SNAP Enclosure 8x10x1.75 Ver1.A\drawings\SNAP Ver2 pack-n-go\Workgroups\NotInProject\RESC1005X35N_R90.ipt
- C:\Users\rtreacy\Documents\Inventor\SNAP Enclosure 8x10x1.75 Ver1.A\drawings\SNAP Ver2 pack-n-go\Workgroups\NotInProject\RESC1005X35N_R93.ipt
- C:\Users\rtreacy\Documents\Inventor\SNAP Enclosure 8x10x1.75 Ver1.A\drawings\SNAP Ver2 pack-n-go\Workgroups\NotInProject\RESC1005X35N_R99.ipt
- C:\Users\rtreacy\Documents\Inventor\SNAP Enclosure 8x10x1.75 Ver1.A\drawings\SNAP Ver2 pack-n-go\Workgroups\NotInProject\RESC1005X35N_R85.ipt
- C:\Users\rtreacy\Documents\Inventor\SNAP Enclosure 8x10x1.75 Ver1.A\drawings\SNAP Ver2 pack-n-go\Workgroups\NotInProject\RESC1005X35N_R87.ipt
- C:\Users\rtreacy\Documents\Inventor\SNAP Enclosure 8x10x1.75 Ver1.A\drawings\SNAP Ver2 pack-n-go\Workgroups\NotInProject\RESC1005X35N_R407.ipt
- C:\Users\rtreacy\Documents\Inventor\SNAP Enclosure 8x10x1.75 Ver1.A\drawings\SNAP Ver2 pack-n-go\Workgroups\NotInProject\RESC1005X35N_R408.ipt
- C:\Users\rtreacy\Documents\Inventor\SNAP Enclosure 8x10x1.75 Ver1.A\drawings\SNAP Ver2 pack-n-go\Workgroups\NotInProject\RESC1608X50N_R441.ipt
- C:\Users\rtreacy\Documents\Inventor\SNAP Enclosure 8x10x1.75 Ver1.A\drawings\SNAP Ver2 pack-n-go\Workgroups\NotInProject\RESC1608X50N_R440.ipt
- C:\Users\rtreacy\Documents\Inventor\SNAP Enclosure 8x10x1.75 Ver1.A\drawings\SNAP Ver2 pack-n-go\Workgroups\NotInProject\RESC1608X50N_R439.ipt
- C:\Users\rtreacy\Documents\Inventor\SNAP Enclosure 8x10x1.75 Ver1.A\drawings\SNAP Ver2 pack-n-go\Workgroups\NotInProject\RESC1608X50N_R435.ipt
- C:\Users\rtreacy\Documents\Inventor\SNAP Enclosure 8x10x1.75 Ver1.A\drawings\SNAP Ver2 pack-n-go\Workgroups\NotInProject\RESC1608X50N_R101.ipt
- C:\Users\rtreacy\Documents\Inventor\SNAP Enclosure 8x10x1.75 Ver1.A\drawings\SNAP Ver2 pack-n-go\Workgroups\NotInProject\RESC1608X50N_R107.ipt
- C:\Users\rtreacy\Documents\Inventor\SNAP Enclosure 8x10x1.75 Ver1.A\drawings\SNAP Ver2 pack-n-go\Workgroups\NotInProject\RESC1608X50N_R108.ipt
- C:\Users\rtreacy\Documents\Inventor\SNAP Enclosure 8x10x1.75 Ver1.A\drawings\SNAP Ver2 pack-n-go\Workgroups\NotInProject\RESC1608X50N_R78.ipt
- C:\Users\rtreacy\Documents\Inventor\SNAP Enclosure 8x10x1.75 Ver1.A\drawings\SNAP Ver2 pack-n-go\Workgroups\NotInProject\RESC1608X50N_R79.ipt
- C:\Users\rtreacy\Documents\Inventor\SNAP Enclosure 8x10x1.75 Ver1.A\drawings\SNAP Ver2 pack-n-go\Workgroups\NotInProject\RESC1608X50N_R88.ipt
- C:\Users\rtreacy\Documents\Inventor\SNAP Enclosure 8x10x1.75 Ver1.A\drawings\SNAP Ver2 pack-n-go\Workgroups\NotInProject\RESC1608X50N_R89.ipt
- C:\Users\rtreacy\Documents\Inventor\SNAP Enclosure 8x10x1.75 Ver1.A\drawings\SNAP Ver2 pack-n-go\Workgroups\NotInProject\RESC1608X50N_R98.ipt
- C:\Users\rtreacy\Documents\Inventor\SNAP Enclosure 8x10x1.75 Ver1.A\drawings\SNAP Ver2 pack-n-go\Workgroups\NotInProject\RESC1608X50N_R192.ipt
- C:\Users\rtreacy\Documents\Inventor\SNAP Enclosure 8x10x1.75 Ver1.A\drawings\SNAP Ver2 pack-n-go\Workgroups\NotInProject\RESC1608X50N_R193.ipt
- C:\Users\rtreacy\Documents\Inventor\SNAP Enclosure 8x10x1.75 Ver1.A\drawings\SNAP Ver2 pack-n-go\Workgroups\NotInProject\RESC1608X50N_R149.ipt
- C:\Users\rtreacy\Documents\Inventor\SNAP Enclosure 8x10x1.75 Ver1.A\drawings\SNAP Ver2 pack-n-go\Workgroups\NotInProject\RESC1608X50N_R153.ipt
- C:\Users\rtreacy\Documents\Inventor\SNAP Enclosure 8x10x1.75 Ver1.A\drawings\SNAP Ver2 pack-n-go\Workgroups\NotInProject\RESC1608X50N_R68.ipt
- C:\Users\rtreacy\Documents\Inventor\SNAP Enclosure 8x10x1.75 Ver1.A\drawings\SNAP Ver2 pack-n-go\Workgroups\NotInProject\RESC1608X50N_R69.ipt